# Autodesk Inventor assembly: 2 Arm
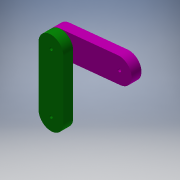
[picture p0: Inventor's stored thumbnail of the model, 180x180]
Saved by Autodesk Inventor 2017 (Build 210142000, 142)
## iProperties
Created: 2017-03-25
Part Number: 2 Arm
Document SubType Name: Assembly
Designer: Parshant Bombhi
Author: Parshant Bombhi
## Documents named in this file (2)
- C:\Users\Parshant Bombhi\sfuvault\Rembrant Robotics\Inventor Files\2 Arm.iam
- C:\Users\Parshant Bombhi\sfuvault\Rembrant Robotics\Inventor Files\Arm.ipt
## Components (2 placed, 1 different names)
1. Arm:1 — Mate:1, Mate:2
2. Arm:2 — Mate:1, Mate:2
## Relationships (2: Mate 2)
- Mate:1: Arm:1 ↔ Arm:2
- Mate:2: Arm:1 ↔ Arm:2
